# Autodesk Inventor assembly: KanawaTsugi
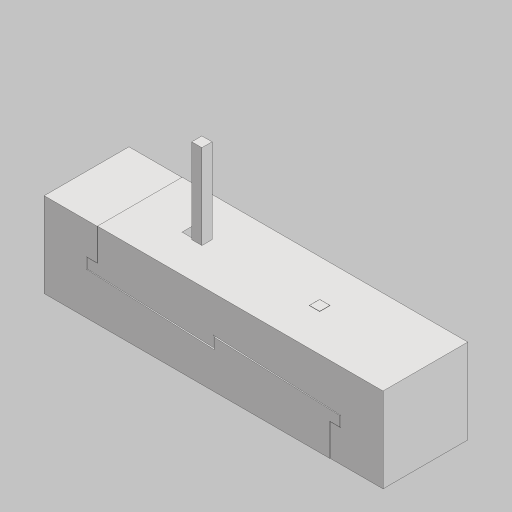
[picture p0: Inventor's stored thumbnail of the model, 512x512]
Saved by Autodesk Inventor 2023 (Build 270158000, 158)
## iProperties
Created: 2026-02-22
Part Number: KanawaTsugi
Document SubType Name: Assembly
Designer: MARTIN MAESTRE
Author: MARTIN MAESTRE
## Documents named in this file (3)
- C:\Users\MARTIN MAESTRE\OneDrive - Universidad de los Andes\POSTGRADO\202610\MAESTRIA\PROBLEMA ESPECIAL\CADS\Fig4\KanawaTsugi.iam
- C:\Users\MARTIN MAESTRE\OneDrive - Universidad de los Andes\POSTGRADO\202610\MAESTRIA\PROBLEMA ESPECIAL\CADS\Fig4\Hembra.ipt
- C:\Users\MARTIN MAESTRE\OneDrive - Universidad de los Andes\POSTGRADO\202610\MAESTRIA\PROBLEMA ESPECIAL\CADS\Fig4\Pines.ipt
## Components (4 placed, 2 different names)
1. Hembra:1 — Coincidencia:1, Coincidencia:2, Coincidencia:3, Coincidencia:4, Nivelación:1, Coincidencia:5
2. Hembra:2 — Coincidencia:4, Nivelación:1
3. Pines:1 — Coincidencia:5
4. Pines:2
## Relationships (6: Mate 5, Flush 1)
- Coincidencia:1 [Mate]: Hembra:1
- Coincidencia:2 [Mate]: Hembra:1
- Coincidencia:3 [Mate]: Hembra:1
- Coincidencia:4 [Mate]: Hembra:1 ↔ Hembra:2
- Nivelación:1 [Flush]: Hembra:1 ↔ Hembra:2
- Coincidencia:5 [Mate]: Hembra:1 ↔ Pines:1
